# Autodesk Inventor assembly: chassi2.0
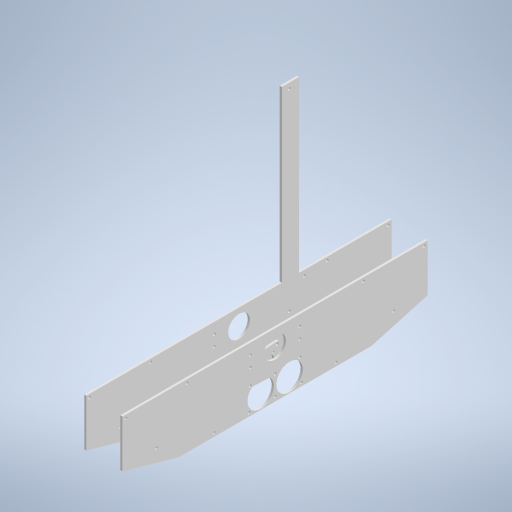
[picture p0: Inventor's stored thumbnail of the model, 512x512]
Saved by Autodesk Inventor 2023 (Build 270158000, 158)
## iProperties
Created: 2022-09-06
Part Number: chassi2.0
Document SubType Name: Assembly
Designer: deli
Author: deli
## Documents named in this file (17)
- C:\Users\deli\OneDrive - Eastside Preparatory School\FTC\8103-power-play\CAD\chassi2.0.iam
- C:\Users\deli\OneDrive - Eastside Preparatory School\FTC\8103-power-play\CAD\Outside Chassi Plate low.ipt
- C:\Users\deli\OneDrive - Eastside Preparatory School\FTC\8103-power-play\CAD\Mecanum Wheel.iam
- C:\Users\deli\OneDrive - Eastside Preparatory School\FTC\8103-power-play\CAD\chassi axel 50mm.ipt
- C:\Users\deli\OneDrive - Eastside Preparatory School\FTC\8103-power-play\CAD\FTC-parts\goBILDA\2802-0004-0010.ipt
- C:\Users\deli\OneDrive - Eastside Preparatory School\FTC\8103-power-play\CAD\Mecanum Wheel_MIR2.iam
- C:\Users\deli\OneDrive - Eastside Preparatory School\FTC\8103-power-play\CAD\FTC-parts\goBILDA\1611-0514-0006.ipt
- C:\Users\deli\OneDrive - Eastside Preparatory School\FTC\8103-power-play\CAD\FTC-parts\goBILDA\5202-0002-0019 part.ipt
- C:\Users\deli\OneDrive - Eastside Preparatory School\FTC\8103-power-play\CAD\FTC-parts\goBILDA\3417-1006-0016 assembly.ipt
- C:\Users\deli\OneDrive - Eastside Preparatory School\FTC\8103-power-play\CAD\motorMountPlate2.0.ipt
- C:\Users\deli\OneDrive - Eastside Preparatory School\FTC\8103-power-play\CAD\1502-0006-0180 cut down.ipt
- C:\Users\deli\OneDrive - Eastside Preparatory School\FTC\8103-power-play\CAD\insideChassiPlate2.0.ipt
- C:\Users\deli\OneDrive - Eastside Preparatory School\FTC\8103-power-play\CAD\FTC-parts\goBILDA\1501-0006-0500.ipt
- C:\Users\deli\OneDrive - Eastside Preparatory School\FTC\8103-power-play\CAD\1501-0006-0320 cut to 31.175mm.ipt
- C:\Users\deli\OneDrive - Eastside Preparatory School\FTC\8103-power-play\CAD\FTC-parts\goBILDA\2802-0004-0030.ipt
- C:\Users\deli\OneDrive - Eastside Preparatory School\FTC\8103-power-play\CAD\FTC-parts\drivetimingbelt77mm.ipt
- C:\Users\deli\OneDrive - Eastside Preparatory School\FTC\8103-power-play\CAD\FTC-parts\goBILDA\2802-0004-0012.ipt
## Components (63 placed, 16 different names)
1. Outside Chassi Plate low:1 — Mate:2, Mate:3, Mate:4, Mate:5, Mate:6, Mate:7, Mate:8, Mate:10, Mate:11, Mate:15, Mate:16, Mate:17, Mate:18, Mate:19, Mate:20, Mate:21, Mate:22, Mate:23, Mate:24, Mate:25, Mate:26, Mate:27, Mate:28, Mate:29, Mate:30, Mate:36, Mate:37, Mate:38, Mate:39, Mate:40, Mate:42, Mate:43, Mate:44, Mate:45, Mate:47, Mate:48, Mate:49, Mate:63, Mate:64, Mate:65, Mate:66, Mate:67, Mate:68, Mate:69, Mate:70, Mate:71, Mate:72, Mate:73, Mate:74, Mate:102, Mate:103, Mate:104, Mate:105, Mate:106, Mate:108, Mate:109, Mate:110, Mate:112, Mate:113, Mate:141, Mate:142, Mate:143
2. Mecanum Wheel:1 [sub-assembly] — Mate:4, Mate:11, Mate:12, Flush:4
3. chassi axel 50mm:1 — Mate:2, Mate:3, Mate:9, Mate:62, Mate:130
4. 2802-0004-0010:1 — Mate:17, Mate:18
5. 2802-0004-0010:2 — Mate:5, Mate:6
6. Mecanum Wheel_MIR2:1 [sub-assembly] — Mate:9, Mate:10, Flush:2, Mate:140
7. chassi axel 50mm:2 — Mate:7, Mate:8, Mate:12, Mate:136
8. 1611-0514-0006:1 — Mate:15, Mate:16
9. 5202-0002-0019 part:1 — Mate:32
10. 3417-1006-0016 assembly:1 — Flush:2, Mate:118, Mate:120
11. motorMountPlate2.0:1 — Mate:32
12. 1502-0006-0180 cut down:1 — Mate:23, Mate:29
13. 1502-0006-0180 cut down:2 — Mate:24, Mate:30
14. 1502-0006-0180 cut down:3 — Mate:22, Mate:28
15. 1502-0006-0180 cut down:4 — Mate:21, Mate:27
16. 1502-0006-0180 cut down:5 — Mate:20, Mate:25
17. 1502-0006-0180 cut down:6 — Mate:19, Mate:26
18. 1611-0514-0006:2 — Mate:36, Mate:37
19. 5202-0002-0019 part:2
20. 3417-1006-0016 assembly:2 — Flush:4, Mate:117
21. insideChassiPlate2.0:1 — Mate:50, Mate:51, Mate:52, Mate:53, Mate:54, Mate:55, Mate:62, Mate:75, Mate:76, Mate:77, Mate:78, Mate:79, Mate:80, Mate:81, Mate:83, Mate:84, Mate:85, Mate:86, Mate:98, Mate:99, Mate:145, Mate:147, Mate:148
22. 1501-0006-0500:1 — Mate:38, Mate:48, Mate:127, Mate:147
23. 1501-0006-0500:3 — Mate:39, Mate:47, Mate:128
24. 1501-0006-0500:4 — Mate:42, Mate:45, Mate:135
25. 1501-0006-0500:5 — Mate:43, Mate:44, Mate:137, Mate:148
26. 1501-0006-0500:6 — Mate:40, Mate:49, Mate:129
27. 1501-0006-0320 cut to 31.175mm:1 — Mate:55, Mate:121, Mate:132
28. 1501-0006-0320 cut to 31.175mm:2 — Mate:54, Mate:124, Mate:131
29. 1501-0006-0320 cut to 31.175mm:3 — Mate:51, Mate:126, Mate:139
30. 1501-0006-0320 cut to 31.175mm:4 — Mate:50, Mate:125, Mate:138
31. 1501-0006-0320 cut to 31.175mm:5 — Mate:53, Mate:122, Mate:133
32. 1501-0006-0320 cut to 31.175mm:6 — Mate:52, Mate:123, Mate:134
33. 2802-0004-0030:1 — Mate:67, Mate:71, Mate:126
34. 2802-0004-0030:2 — Mate:66, Mate:70, Mate:122
35. 2802-0004-0030:3 — Mate:65, Mate:72, Mate:125
36. 2802-0004-0030:4 — Mate:63, Mate:73, Mate:121
37. 2802-0004-0030:5 — Mate:64, Mate:74, Mate:124
38. 2802-0004-0030:6 — Mate:68, Mate:69, Mate:123
39. 2802-0004-0010:3 — Mate:86, Mate:130
40. 2802-0004-0010:4 — Mate:85, Mate:131
41. 2802-0004-0010:5 — Mate:84, Mate:137
42. 2802-0004-0010:6 — Mate:83, Mate:139
43. 2802-0004-0010:7 — Mate:81, Mate:138
44. 2802-0004-0010:8 — Mate:80, Mate:133
45. 2802-0004-0010:10 — Mate:78, Mate:127
46. 2802-0004-0010:11 — Mate:77, Mate:136
47. 2802-0004-0010:12 — Mate:79, Mate:135
48. 2802-0004-0010:13 — Mate:75, Mate:134
49. 2802-0004-0010:14 — Mate:76, Mate:132
50. 2802-0004-0010:15 — Mate:98, Mate:128
51. 2802-0004-0010:16 — Mate:99, Mate:129
52. 2802-0004-0010:17 — Mate:108, Mate:109
53. 2802-0004-0010:19 — Mate:106, Mate:110
54. 2802-0004-0010:20 — Mate:104, Mate:112
55. 2802-0004-0010:21 — Mate:102, Mate:103
56. 2802-0004-0010:22 — Mate:105, Mate:113
57. drivetimingbelt77mm:1 — Mate:117
58. drivetimingbelt77mm:2 — Mate:118, Mate:120, Mate:140
59. 2802-0004-0010:23 — Mate:141, Mate:142, Mate:144
60. 1501-0006-0500:7 — Mate:143, Mate:144, Mate:146
61. 2802-0004-0010:24 — Mate:145, Mate:146
62. 2802-0004-0012:2
63. 2802-0004-0012:1
## Relationships (125: Mate 121, Flush 4)
- Mate:2: Outside Chassi Plate low:1 ↔ chassi axel 50mm:1
- Mate:3: Outside Chassi Plate low:1 ↔ chassi axel 50mm:1
- Mate:4: Outside Chassi Plate low:1 ↔ Mecanum Wheel:1
- Mate:5: Outside Chassi Plate low:1 ↔ 2802-0004-0010:2
- Mate:6: Outside Chassi Plate low:1 ↔ 2802-0004-0010:2
- Mate:7: Outside Chassi Plate low:1 ↔ chassi axel 50mm:2
- Mate:8: Outside Chassi Plate low:1 ↔ chassi axel 50mm:2
- Mate:9: chassi axel 50mm:1 ↔ Mecanum Wheel_MIR2:1
- Mate:10: Outside Chassi Plate low:1 ↔ Mecanum Wheel_MIR2:1
- Mate:11: Outside Chassi Plate low:1 ↔ Mecanum Wheel:1
- Mate:12: Mecanum Wheel:1 ↔ chassi axel 50mm:2
- [Mate]: 1611-0514-0006:1 ↔ 5202-0002-0019 part:1
- [Flush]: 1611-0514-0006:1 ↔ 5202-0002-0019 part:1
- [Mate]: 5202-0002-0019 part:1 ↔ 3417-1006-0016 assembly:1
- Mate:15: Outside Chassi Plate low:1 ↔ 1611-0514-0006:1
- Mate:16: Outside Chassi Plate low:1 ↔ 1611-0514-0006:1
- Flush:2: Mecanum Wheel_MIR2:1 ↔ 3417-1006-0016 assembly:1
- Mate:17: Outside Chassi Plate low:1 ↔ 2802-0004-0010:1
- Mate:18: Outside Chassi Plate low:1 ↔ 2802-0004-0010:1
- Mate:19: Outside Chassi Plate low:1 ↔ 1502-0006-0180 cut down:6
- Mate:20: Outside Chassi Plate low:1 ↔ 1502-0006-0180 cut down:5
- Mate:21: Outside Chassi Plate low:1 ↔ 1502-0006-0180 cut down:4
- Mate:22: Outside Chassi Plate low:1 ↔ 1502-0006-0180 cut down:3
- Mate:23: Outside Chassi Plate low:1 ↔ 1502-0006-0180 cut down:1
- Mate:24: Outside Chassi Plate low:1 ↔ 1502-0006-0180 cut down:2
- Mate:25: Outside Chassi Plate low:1 ↔ 1502-0006-0180 cut down:5
- Mate:26: Outside Chassi Plate low:1 ↔ 1502-0006-0180 cut down:6
- Mate:27: Outside Chassi Plate low:1 ↔ 1502-0006-0180 cut down:4
- Mate:28: Outside Chassi Plate low:1 ↔ 1502-0006-0180 cut down:3
- Mate:29: Outside Chassi Plate low:1 ↔ 1502-0006-0180 cut down:1
- Mate:30: Outside Chassi Plate low:1 ↔ 1502-0006-0180 cut down:2
- Mate:32: 5202-0002-0019 part:1 ↔ motorMountPlate2.0:1
- [Mate]: 1611-0514-0006:2 ↔ 5202-0002-0019 part:2
- [Flush]: 1611-0514-0006:2 ↔ 5202-0002-0019 part:2
- [Mate]: 5202-0002-0019 part:2 ↔ 3417-1006-0016 assembly:2
- Mate:36: Outside Chassi Plate low:1 ↔ 1611-0514-0006:2
- Mate:37: Outside Chassi Plate low:1 ↔ 1611-0514-0006:2
- Flush:4: Mecanum Wheel:1 ↔ 3417-1006-0016 assembly:2
- Mate:38: Outside Chassi Plate low:1 ↔ 1501-0006-0500:1
- Mate:39: Outside Chassi Plate low:1 ↔ 1501-0006-0500:3
- Mate:40: Outside Chassi Plate low:1 ↔ 1501-0006-0500:6
- Mate:42: Outside Chassi Plate low:1 ↔ 1501-0006-0500:4
- Mate:43: Outside Chassi Plate low:1 ↔ 1501-0006-0500:5
- Mate:44: Outside Chassi Plate low:1 ↔ 1501-0006-0500:5
- Mate:45: Outside Chassi Plate low:1 ↔ 1501-0006-0500:4
- Mate:47: Outside Chassi Plate low:1 ↔ 1501-0006-0500:3
- Mate:48: Outside Chassi Plate low:1 ↔ 1501-0006-0500:1
- Mate:49: Outside Chassi Plate low:1 ↔ 1501-0006-0500:6
- Mate:50: insideChassiPlate2.0:1 ↔ 1501-0006-0320 cut to 31.175mm:4
- Mate:51: insideChassiPlate2.0:1 ↔ 1501-0006-0320 cut to 31.175mm:3
- Mate:52: insideChassiPlate2.0:1 ↔ 1501-0006-0320 cut to 31.175mm:6
- Mate:53: insideChassiPlate2.0:1 ↔ 1501-0006-0320 cut to 31.175mm:5
- Mate:54: insideChassiPlate2.0:1 ↔ 1501-0006-0320 cut to 31.175mm:2
- Mate:55: insideChassiPlate2.0:1 ↔ 1501-0006-0320 cut to 31.175mm:1
- Mate:62: chassi axel 50mm:1 ↔ insideChassiPlate2.0:1
- Mate:63: Outside Chassi Plate low:1 ↔ 2802-0004-0030:4
- Mate:64: Outside Chassi Plate low:1 ↔ 2802-0004-0030:5
- Mate:65: Outside Chassi Plate low:1 ↔ 2802-0004-0030:3
- Mate:66: Outside Chassi Plate low:1 ↔ 2802-0004-0030:2
- Mate:67: Outside Chassi Plate low:1 ↔ 2802-0004-0030:1
- Mate:68: Outside Chassi Plate low:1 ↔ 2802-0004-0030:6
- Mate:69: Outside Chassi Plate low:1 ↔ 2802-0004-0030:6
- Mate:70: Outside Chassi Plate low:1 ↔ 2802-0004-0030:2
- Mate:71: Outside Chassi Plate low:1 ↔ 2802-0004-0030:1
- Mate:72: Outside Chassi Plate low:1 ↔ 2802-0004-0030:3
- Mate:73: Outside Chassi Plate low:1 ↔ 2802-0004-0030:4
- Mate:74: Outside Chassi Plate low:1 ↔ 2802-0004-0030:5
- Mate:75: insideChassiPlate2.0:1 ↔ 2802-0004-0010:13
- Mate:76: insideChassiPlate2.0:1 ↔ 2802-0004-0010:14
- Mate:77: insideChassiPlate2.0:1 ↔ 2802-0004-0010:11
- Mate:78: insideChassiPlate2.0:1 ↔ 2802-0004-0010:10
- Mate:79: insideChassiPlate2.0:1 ↔ 2802-0004-0010:12
- Mate:80: insideChassiPlate2.0:1 ↔ 2802-0004-0010:8
- Mate:81: insideChassiPlate2.0:1 ↔ 2802-0004-0010:7
- Mate:83: insideChassiPlate2.0:1 ↔ 2802-0004-0010:6
- Mate:84: insideChassiPlate2.0:1 ↔ 2802-0004-0010:5
- Mate:85: insideChassiPlate2.0:1 ↔ 2802-0004-0010:4
- Mate:86: insideChassiPlate2.0:1 ↔ 2802-0004-0010:3
- Mate:98: insideChassiPlate2.0:1 ↔ 2802-0004-0010:15
- Mate:99: insideChassiPlate2.0:1 ↔ 2802-0004-0010:16
- Mate:102: Outside Chassi Plate low:1 ↔ 2802-0004-0010:21
- Mate:103: Outside Chassi Plate low:1 ↔ 2802-0004-0010:21
- Mate:104: Outside Chassi Plate low:1 ↔ 2802-0004-0010:20
- Mate:105: Outside Chassi Plate low:1 ↔ 2802-0004-0010:22
- Mate:106: Outside Chassi Plate low:1 ↔ 2802-0004-0010:19
- Mate:108: Outside Chassi Plate low:1 ↔ 2802-0004-0010:17
- Mate:109: Outside Chassi Plate low:1 ↔ 2802-0004-0010:17
- Mate:110: Outside Chassi Plate low:1 ↔ 2802-0004-0010:19
- Mate:112: Outside Chassi Plate low:1 ↔ 2802-0004-0010:20
- Mate:113: Outside Chassi Plate low:1 ↔ 2802-0004-0010:22
- Mate:117 (0.125 mm): 3417-1006-0016 assembly:2 ↔ drivetimingbelt77mm:1
- Mate:118: 3417-1006-0016 assembly:1 ↔ drivetimingbelt77mm:2
- Mate:120 (0.125 mm): 3417-1006-0016 assembly:1 ↔ drivetimingbelt77mm:2
- Mate:121: 1501-0006-0320 cut to 31.175mm:1 ↔ 2802-0004-0030:4
- Mate:122: 1501-0006-0320 cut to 31.175mm:5 ↔ 2802-0004-0030:2
- Mate:123: 1501-0006-0320 cut to 31.175mm:6 ↔ 2802-0004-0030:6
- Mate:124: 1501-0006-0320 cut to 31.175mm:2 ↔ 2802-0004-0030:5
- Mate:125: 1501-0006-0320 cut to 31.175mm:4 ↔ 2802-0004-0030:3
- Mate:126: 1501-0006-0320 cut to 31.175mm:3 ↔ 2802-0004-0030:1
- Mate:127: 1501-0006-0500:1 ↔ 2802-0004-0010:10
- Mate:128: 1501-0006-0500:3 ↔ 2802-0004-0010:15
- Mate:129: 1501-0006-0500:6 ↔ 2802-0004-0010:16
- Mate:130: chassi axel 50mm:1 ↔ 2802-0004-0010:3
- Mate:131: 1501-0006-0320 cut to 31.175mm:2 ↔ 2802-0004-0010:4
- Mate:132: 1501-0006-0320 cut to 31.175mm:1 ↔ 2802-0004-0010:14
- Mate:133: 1501-0006-0320 cut to 31.175mm:5 ↔ 2802-0004-0010:8
- Mate:134: 1501-0006-0320 cut to 31.175mm:6 ↔ 2802-0004-0010:13
- Mate:135: 1501-0006-0500:4 ↔ 2802-0004-0010:12
- Mate:136: chassi axel 50mm:2 ↔ 2802-0004-0010:11
- Mate:137: 1501-0006-0500:5 ↔ 2802-0004-0010:5
- Mate:138: 1501-0006-0320 cut to 31.175mm:4 ↔ 2802-0004-0010:7
- Mate:139: 1501-0006-0320 cut to 31.175mm:3 ↔ 2802-0004-0010:6
- Mate:140: Mecanum Wheel_MIR2:1 ↔ drivetimingbelt77mm:2
- Mate:141: Outside Chassi Plate low:1 ↔ 2802-0004-0010:23
- Mate:142: Outside Chassi Plate low:1 ↔ 2802-0004-0010:23
- Mate:143: Outside Chassi Plate low:1 ↔ 1501-0006-0500:7
- Mate:144: 2802-0004-0010:23 ↔ 1501-0006-0500:7
- Mate:145: insideChassiPlate2.0:1 ↔ 2802-0004-0010:24
- Mate:146: 1501-0006-0500:7 ↔ 2802-0004-0010:24
- Mate:147: insideChassiPlate2.0:1 ↔ 1501-0006-0500:1
- Mate:148: insideChassiPlate2.0:1 ↔ 1501-0006-0500:5
- [Mate]: Outside Chassi Plate low:1 ↔ 2802-0004-0012:1
- [Mate]: Outside Chassi Plate low:1 ↔ 2802-0004-0012:1
- [Mate]: Outside Chassi Plate low:1 ↔ 2802-0004-0012:2
- [Mate]: Outside Chassi Plate low:1 ↔ 2802-0004-0012:2
## Named parameters: d34_d47 = 0 mm, d35_d48 = 0 mm, d36_d64 = 0 mm
